# Autodesk Inventor assembly: PocketPoint
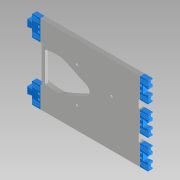
[picture p0: Inventor's stored thumbnail of the model, 180x180]
Saved by Autodesk Inventor 2021 (Build 250183000, 183)
## iProperties
Created: 2021-03-05
Part Number: PocketPoint
Document SubType Name: Assembly
Designer: kumagai
Author: kumagai
## Documents named in this file (4)
- X:\Develop\CAD\PlaRails\PocketTrackPoint\PocketPoint.iam
- X:\Develop\CAD\PlaRails\PocketTrackPoint\PocketPoint.ipt
- X:\Develop\CAD\PlaRails\RailJointFemale.ipt
- X:\Develop\CAD\PlaRails\RailJointMale.ipt
## Components (6 placed, 3 different names)
1. PocketPoint:1 — フラッシュ:1, フラッシュ:2, フラッシュ:3, フラッシュ:4, フラッシュ:5, メイト:1, メイト:2, メイト:3, メイト:4, メイト:5, フラッシュ:6, フラッシュ:7, フラッシュ:8, フラッシュ:9, フラッシュ:10
2. RailJointFemale:1 — フラッシュ:5, メイト:5, フラッシュ:9
3. RailJointFemale:2 — フラッシュ:3, メイト:3, フラッシュ:7
4. RailJointFemale:3 — フラッシュ:4, メイト:4, フラッシュ:10
5. RailJointMale:1 — フラッシュ:2, メイト:2, フラッシュ:8
6. RailJointMale:2 — フラッシュ:1, メイト:1, フラッシュ:6
## Relationships (15: Flush 10, Mate 5)
- フラッシュ:1 [Flush]: PocketPoint:1 ↔ RailJointMale:2
- フラッシュ:2 [Flush]: PocketPoint:1 ↔ RailJointMale:1
- フラッシュ:3 [Flush]: PocketPoint:1 ↔ RailJointFemale:2
- フラッシュ:4 [Flush]: PocketPoint:1 ↔ RailJointFemale:3
- フラッシュ:5 [Flush]: PocketPoint:1 ↔ RailJointFemale:1
- メイト:1 [Mate]: PocketPoint:1 ↔ RailJointMale:2
- メイト:2 [Mate]: PocketPoint:1 ↔ RailJointMale:1
- メイト:3 [Mate]: PocketPoint:1 ↔ RailJointFemale:2
- メイト:4 [Mate]: PocketPoint:1 ↔ RailJointFemale:3
- メイト:5 [Mate]: PocketPoint:1 ↔ RailJointFemale:1
- フラッシュ:6 [Flush]: PocketPoint:1 ↔ RailJointMale:2
- フラッシュ:7 [Flush]: PocketPoint:1 ↔ RailJointFemale:2
- フラッシュ:8 [Flush]: PocketPoint:1 ↔ RailJointMale:1
- フラッシュ:9 [Flush]: PocketPoint:1 ↔ RailJointFemale:1
- フラッシュ:10 [Flush]: PocketPoint:1 ↔ RailJointFemale:3
